# Autodesk Inventor assembly: AM14U3 Square Half
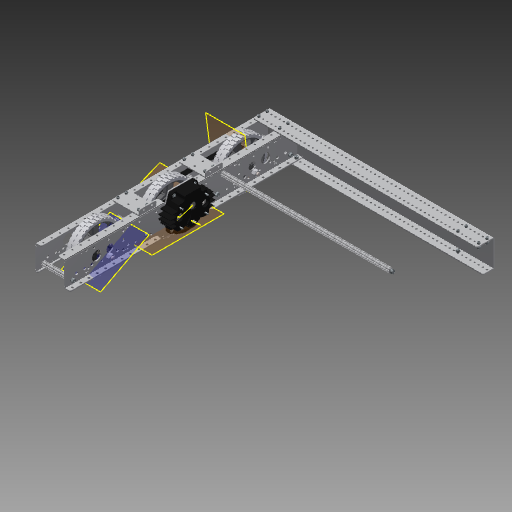
[picture p0: Inventor's stored thumbnail of the model, 512x512]
Saved by Autodesk Inventor 2017.1 (Build 211199000, 199)
## iProperties
Created: 2015-12-07
Part Number: AM14U3 Square Half
Document SubType Name: Assembly
Designer: PhillipD
Author: PhillipD
Revision Number: ANY
## Documents named in this file (9)
- D:\FIRST\FIRST KOP 2017\FIRST Drive Base\Parts\AM14U3 Square Half.iam
- D:\FIRST\FIRST KOP 2017\FIRST Drive Base\Parts\AM14U3 Square Frame Half.iam
- D:\FIRST\FIRST KOP 2017\FIRST Drive Base\Parts\am-2598_107 2016 KOP Toughbox Mini.iam
- D:\FIRST\FIRST KOP 2017\FIRST Drive Base\Parts\6 HiGrip with hub and double pulley.iam
- D:\FIRST\FIRST KOP 2017\FIRST Drive Base\Parts\6 HiGrip with bearings, pulleys and spacers.iam
- D:\FIRST\FIRST KOP 2017\FIRST Drive Base\Parts\FR8ZZ Hex Bearing.ipt
- D:\FIRST\FIRST KOP 2017\FIRST Drive Base\Parts\375-16 x 4.25 Hex Bolt_HFBOLT 0.375-16x2.5x1-C.ipt
- D:\FIRST\FIRST KOP 2017\FIRST Drive Base\Parts\375-16 Lock Nut_91831A127.ipt
- D:\FIRST\FIRST KOP 2017\FIRST Drive Base\Parts\am-2571 655-5M-15 Timing Belt.ipt
## Components (12 placed, 12 different names)
1. AM14U3 Square Frame Half_3 [sub-assembly] — Insert:1, Insert:2, Insert:3
2. am-2598_107 2016 KOP Toughbox Mini_4 [sub-assembly] — Angle:1, Mate:1, Insert:4
3. 6 HiGrip with hub and double pulley_5 [sub-assembly] — Angle:1, Insert:4
4. 6 HiGrip with bearings, pulleys and spacers_6 [sub-assembly] — Insert:1
5. 6 HiGrip with bearings, pulleys and spacers_7 [sub-assembly] — Insert:2
6. FR8ZZ Hex Bearing_8 — Insert:3, Mate:1
7. 375-16 x 4.25 Hex Bolt_HFBOLT 0.375-16x2.5x1-C_9
8. 375-16 x 4.25 Hex Bolt_HFBOLT 0.375-16x2.5x1-C_10
9. 375-16 Lock Nut_91831A127_11
10. 375-16 Lock Nut_91831A127_12
11. am-2571 655-5M-15 Timing Belt_13
12. am-2571 655-5M-15 Timing Belt_14
## Relationships (6: Insert 4, Angle 1, Mate 1)
- Insert:1 (0.0762 mm): AM14U3 Square Frame Half_3 ↔ 6 HiGrip with bearings, pulleys and spacers_6
- Insert:2 (0.0762 mm): AM14U3 Square Frame Half_3 ↔ 6 HiGrip with bearings, pulleys and spacers_7
- Angle:1 (0 deg): am-2598_107 2016 KOP Toughbox Mini_4 ↔ 6 HiGrip with hub and double pulley_5
- Insert:3: AM14U3 Square Frame Half_3 ↔ FR8ZZ Hex Bearing_8
- Mate:1: am-2598_107 2016 KOP Toughbox Mini_4 ↔ FR8ZZ Hex Bearing_8
- Insert:4 (0.8128 mm): am-2598_107 2016 KOP Toughbox Mini_4 ↔ 6 HiGrip with hub and double pulley_5
